# Autodesk Inventor assembly: Full Controller
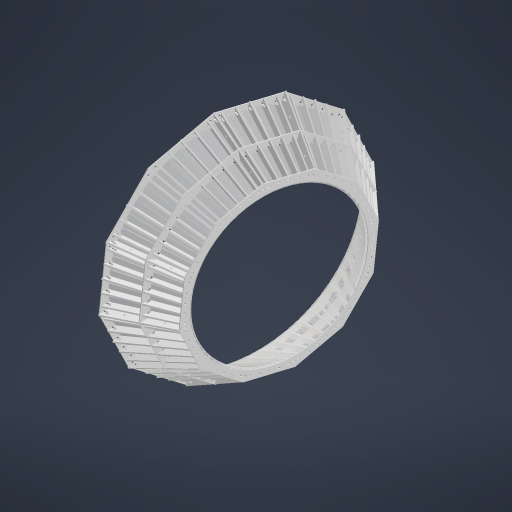
[picture p0: Inventor's stored thumbnail of the model, 512x512]
Saved by Autodesk Inventor 2023 (Build 270158000, 158)
## iProperties
Created: 2022-06-13
Part Number: Full Controller
Document SubType Name: Assembly
Designer: FizzyApple12
Author: FizzyApple12
## Documents named in this file (2)
- C:\Users\FizzyApple12\Desktop\Wacca Controller V3\Full Controller.iam
- C:\Users\FizzyApple12\Desktop\Wacca Controller V3\Half Ring\Half Ring.iam
## Components (2 placed, 1 different names)
1. Half Ring:1 [sub-assembly] — Mate:1, Mate:2
2. Half Ring:2 [sub-assembly] — Mate:1, Mate:2
## Relationships (2: Mate 2)
- Mate:1: Half Ring:1 ↔ Half Ring:2
- Mate:2: Half Ring:1 ↔ Half Ring:2
